# Autodesk Inventor assembly: Circuit à bille
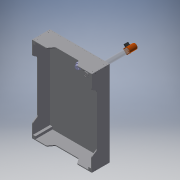
[picture p0: Inventor's stored thumbnail of the model, 180x180]
Saved by Autodesk Inventor 2016 SP1 (Build 200210100, 210)
## iProperties
Created: 2017-04-26
Part Number: Circuit à bille
Material: Générique
Document SubType Name: Assembly
Designer: dimercur
Author: dimercur
## Documents named in this file (9)
- D:\Users\dimercur\Documents\git\dev-gei\dev-gei2\Circuit-a-Bille\Circuit à bille.iam
- D:\Users\dimercur\Documents\git\dev-gei\dev-gei2\Circuit-a-Bille\Caisson.iam
- D:\Users\dimercur\Documents\git\dev-gei\dev-gei2\Circuit-a-Bille\Tube Lanceur.ipt
- D:\Users\dimercur\Documents\git\dev-gei\dev-gei2\Circuit-a-Bille\Pieces importées\Turbine - RV 40 9592506004_CKB_001_-.ipt
- D:\Users\dimercur\Documents\git\dev-gei\dev-gei2\Circuit-a-Bille\Pieces importées\tampon_fj.iam
- D:\Users\dimercur\Documents\git\dev-gei\dev-gei2\Circuit-a-Bille\Pieces importées\te_tj188.ipt
- D:\Users\dimercur\Documents\git\dev-gei\dev-gei2\Circuit-a-Bille\Trappe Lancement.iam
- D:\Users\dimercur\Documents\Inventor\Content Center Files\R2016\fr-FR\ANSI B18.6.4(17)\ANSI B18.6.4 - 8-18 - 3(2) AB II.ipt
- D:\Users\dimercur\Documents\git\dev-gei\dev-gei2\Circuit-a-Bille\Trappe Haute.iam
## Components (9 placed, 8 different names)
1. Caisson:1 [sub-assembly] — Placage:3, Placage:5, Placage:7, Angle:1
2. Tube Lanceur:1 — Cylindrique:1, Placage:8, Cylindrique:2, Placage:9
3. Turbine - RV 40 9592506004_CKB_001_-:1 — Placage:5
4. tampon_fj:1 [sub-assembly] — Placage:6
5. te_tj188:1 — Placage:3, Placage:6, Cylindrique:1, Placage:8
6. Trappe Lancement:1 [sub-assembly] — Placage:7, Angle:1, Logement:1, Logement:2
7. Vis à tôle à tête bombée à empreinte cruciforme - Type AB - Type II N° 8 - 18 - 3:1 — Logement:1
8. Vis à tôle à tête bombée à empreinte cruciforme - Type AB - Type II N° 8 - 18 - 3:2 — Logement:2
9. Trappe Haute:1 [sub-assembly] — Cylindrique:2, Placage:9
## Relationships (11: Mate 6, Insert 2, CylindricalJoint 2, Angle 1)
- Placage:3 [Mate]: Caisson:1 ↔ te_tj188:1
- Placage:5 [Mate] (42 mm): Caisson:1 ↔ Turbine - RV 40 9592506004_CKB_001_-:1
- Placage:6 [Mate]: tampon_fj:1 ↔ te_tj188:1
- Placage:7 [Mate]: Caisson:1 ↔ Trappe Lancement:1
- Angle:1 (0 deg): Caisson:1 ↔ Trappe Lancement:1
- Logement:1 [Insert]: Trappe Lancement:1 ↔ Vis à tôle à tête bombée à empreinte cruciforme - Type AB - Type II N° 8 - 18 - 3:1
- Logement:2 [Insert]: Trappe Lancement:1 ↔ Vis à tôle à tête bombée à empreinte cruciforme - Type AB - Type II N° 8 - 18 - 3:2
- Cylindrique:1: Tube Lanceur:1 ↔ te_tj188:1
- Placage:8 [Mate]: Tube Lanceur:1 ↔ te_tj188:1
- Cylindrique:2: Tube Lanceur:1 ↔ Trappe Haute:1
- Placage:9 [Mate]: Tube Lanceur:1 ↔ Trappe Haute:1
